# Autodesk Inventor assembly: Enclosure02
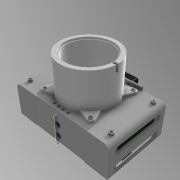
[picture p0: Inventor's stored thumbnail of the model, 180x180]
Saved by Autodesk Inventor 2013 (Build 170138000, 138)
## iProperties
Created: 2014-04-13
Part Number: Enclosure02
Document SubType Name: Assembly
Designer: spichelh
Author: spichelh
## Documents named in this file (22)
- C:\Users\spichelh\Documents\GitHub\beta-hardware\Enclosure\Version 002\Enclosure02.iam
- C:\Users\spichelh\Documents\GitHub\beta-hardware\Enclosure\Version 002\PCB01.ipt
- C:\Users\spichelh\Documents\GitHub\beta-hardware\Enclosure\Version 002\Microzed01.ipt
- C:\Users\spichelh\Documents\GitHub\beta-hardware\Enclosure\Version 002\AddonPCB01.ipt
- C:\Users\spichelh\Documents\GitHub\beta-hardware\Enclosure\Version 002\Enclosure-Backplate01.ipt
- C:\Users\spichelh\Documents\GitHub\beta-hardware\Enclosure\Version 002\KAC12040.ipt
- C:\Users\spichelh\Documents\GitHub\beta-hardware\Enclosure\Version 002\IRGlass.ipt
- C:\Users\spichelh\Documents\GitHub\beta-hardware\Enclosure\Version 002\Cooler.ipt
- C:\Users\spichelh\Documents\GitHub\beta-hardware\Enclosure\Version 002\Nikon Mount 02.ipt
- C:\Users\spichelh\Documents\GitHub\beta-hardware\Enclosure\Version 002\IOModulePlate01.ipt
- C:\Users\spichelh\Documents\GitHub\beta-hardware\Enclosure\Version 002\PCBModuleLeft01.ipt
- C:\Users\spichelh\Documents\GitHub\beta-hardware\Enclosure\Version 002\IOModulePlate02.ipt
- C:\Users\spichelh\Documents\GitHub\beta-hardware\Enclosure\Version 002\IOModulePlate03.ipt
- C:\Users\spichelh\Documents\GitHub\beta-hardware\Enclosure\Version 002\PCBModuleRight01.ipt
- C:\Users\spichelh\Documents\GitHub\beta-hardware\Enclosure\Version 002\LensBase02.ipt
- C:\Users\spichelh\Documents\GitHub\beta-hardware\Enclosure\Version 002\HexSaver01.ipt
- C:\Users\spichelh\Documents\GitHub\beta-hardware\Enclosure\Version 002\Enclosure03.ipt
- C:\Users\spichelh\Documents\Inventor\Content Center Files\R2013\en-US\ANSI B18.3.1M(1)\ANSI B18.3.1M - M2,5x0,45 x 16(2).ipt
- C:\Users\spichelh\Documents\Inventor\Content Center Files\R2013\en-US\ANSI B18.3.1M(1)\ANSI B18.3.1M - M2,5x0,45 x 35(2).ipt
- C:\Users\spichelh\Documents\GitHub\beta-hardware\Enclosure\Version 002\LensBaseTop01.ipt
- C:\Users\spichelh\Documents\Inventor\Content Center Files\R2013\en-US\ANSI B18.6.3(00)\ANSI B18.6.3 - 3-48 UNC - 0,25(32).ipt
- C:\Users\spichelh\Documents\GitHub\beta-hardware\Enclosure\Version 002\Unmate01.ipt
## Components (34 placed, 21 different names)
1. Enclosure03:1 — Flush:26, Mate:33, Mate:34, Mate:38, Flush:40, Mate:39, Insert:9, Insert:10, Insert:11, Insert:13, Insert:14, Insert:26, Insert:27, Insert:28, Insert:29
2. PCB01:1 — Mate:1, Flush:1, Flush:2, Flush:21, Flush:22, Flush:23, Insert:1, Mate:37, Flush:41, Flush:42, Mate:40, Mate:41, Mate:42, Mate:43, Mate:44, Mate:45, Insert:15, Mate:46, Mate:47, Insert:16, Mate:48, Mate:49, Insert:17, Mate:64, Mate:62, Mate:65, Mate:58, Mate:56
3. Microzed01:1 — Mate:1, Flush:1, Flush:2, Flush:22, Flush:24, Flush:27, Mate:36
4. AddonPCB01:1 — Flush:24, Flush:27, Mate:36
5. Enclosure-Backplate01:1 — Mate:38, Flush:40
6. KAC12040:1 — Mate:37
7. IRGlass:1 — Mate:50, Mate:51, Mate:52
8. Cooler:1 — Mate:35, Flush:43, Flush:44, Mate:67, Mate:68, Mate:69
9. Nikon Mount 02:1 — Mate:31, Mate:32, Insert:3, Mate:50, Mate:51, Mate:52, Insert:18, Insert:19, Insert:20, Insert:21
10. LensBase02:1 — Mate:31, Mate:32, Insert:1, Flush:26, Mate:33, Mate:34, Insert:3, Mate:35, Flush:43, Flush:44, Flush:45
11. IOModulePlate01:1 — Insert:13, Insert:14
12. PCBModuleLeft01:1 — Flush:21, Flush:23, Mate:62
13. PCBModuleRight01:1 — Flush:41, Flush:42, Mate:40
14. IOModulePlate02:1 — Insert:11
15. IOModulePlate03:1 — Insert:9, Insert:10
16. HexSaver01:1 — Mate:41, Mate:42, Mate:43
17. HexSaver01:2 — Mate:44, Mate:45, Insert:15
18. HexSaver01:3 — Mate:46, Mate:47, Insert:16
19. HexSaver01:4 — Mate:48, Mate:49, Insert:17
20. Broached Socket Head Cap Screw - Metric M2,5x0,45 x 16:1 — Insert:18
21. Broached Socket Head Cap Screw - Metric M2,5x0,45 x 16:2 — Insert:19
22. Broached Socket Head Cap Screw - Metric M2,5x0,45 x 16:3 — Insert:20
23. Broached Socket Head Cap Screw - Metric M2,5x0,45 x 16:4 — Insert:21
24. LensBaseTop01:1 — Flush:45, Mate:53, Mate:54, Mate:67, Mate:68, Mate:69
25. Cross Recessed 100° Flat Countersunk Head Machine Screw - Type I - Inch 3-48 UNC x 0,25:2 — Mate:53
26. Cross Recessed 100° Flat Countersunk Head Machine Screw - Type I - Inch 3-48 UNC x 0,25:1 — Mate:54
27. Broached Socket Head Cap Screw - Metric M2,5x0,45 x 35:5 — Insert:26, Mate:55
28. Broached Socket Head Cap Screw - Metric M2,5x0,45 x 35:6 — Insert:27, Mate:59
29. Broached Socket Head Cap Screw - Metric M2,5x0,45 x 35:7 — Insert:28, Mate:66
30. Broached Socket Head Cap Screw - Metric M2,5x0,45 x 35:8 — Insert:29, Mate:57
31. Unmate01:1 — Mate:55, Mate:56
32. Unmate01:2 — Mate:57, Mate:58
33. Unmate01:3 — Mate:59, Mate:64
34. Unmate01:4 — Mate:65, Mate:66
## Relationships (69: Mate 37, Insert 18, Flush 14)
- Mate:1 (5 mm): PCB01:1 ↔ Microzed01:1
- Flush:1: PCB01:1 ↔ Microzed01:1
- Flush:2: PCB01:1 ↔ Microzed01:1
- Flush:21: PCB01:1 ↔ PCBModuleLeft01:1
- Flush:22: PCB01:1 ↔ Microzed01:1
- Flush:23: PCB01:1 ↔ PCBModuleLeft01:1
- Flush:24: Microzed01:1 ↔ AddonPCB01:1
- Mate:31: Nikon Mount 02:1 ↔ LensBase02:1
- Mate:32: Nikon Mount 02:1 ↔ LensBase02:1
- Insert:1: PCB01:1 ↔ LensBase02:1
- Flush:26: Enclosure03:1 ↔ LensBase02:1
- Mate:33: Enclosure03:1 ↔ LensBase02:1
- Mate:34: Enclosure03:1 ↔ LensBase02:1
- Insert:3: Nikon Mount 02:1 ↔ LensBase02:1
- Mate:35: Cooler:1 ↔ LensBase02:1
- Flush:27: Microzed01:1 ↔ AddonPCB01:1
- Mate:36 (10 mm): Microzed01:1 ↔ AddonPCB01:1
- Mate:37: PCB01:1 ↔ KAC12040:1
- Mate:38 (-1 mm): Enclosure03:1 ↔ Enclosure-Backplate01:1
- Flush:40: Enclosure03:1 ↔ Enclosure-Backplate01:1
- Mate:39: Enclosure03:1
- Flush:41: PCB01:1 ↔ PCBModuleRight01:1
- Flush:42: PCB01:1 ↔ PCBModuleRight01:1
- Mate:40 (6 mm): PCB01:1 ↔ PCBModuleRight01:1
- Insert:9: Enclosure03:1 ↔ IOModulePlate03:1
- Insert:10: Enclosure03:1 ↔ IOModulePlate03:1
- Insert:11: Enclosure03:1 ↔ IOModulePlate02:1
- Insert:13: Enclosure03:1 ↔ IOModulePlate01:1
- Insert:14: Enclosure03:1 ↔ IOModulePlate01:1
- Mate:41: PCB01:1 ↔ HexSaver01:1
- Mate:42: PCB01:1 ↔ HexSaver01:1
- Mate:43: PCB01:1 ↔ HexSaver01:1
- Mate:44: PCB01:1 ↔ HexSaver01:2
- Mate:45: PCB01:1 ↔ HexSaver01:2
- Insert:15: PCB01:1 ↔ HexSaver01:2
- Mate:46: PCB01:1 ↔ HexSaver01:3
- Mate:47: PCB01:1 ↔ HexSaver01:3
- Insert:16: PCB01:1 ↔ HexSaver01:3
- Mate:48: PCB01:1 ↔ HexSaver01:4
- Mate:49: PCB01:1 ↔ HexSaver01:4
- Insert:17: PCB01:1 ↔ HexSaver01:4
- Mate:50: IRGlass:1 ↔ Nikon Mount 02:1
- Mate:51 (0.5 mm): IRGlass:1 ↔ Nikon Mount 02:1
- Mate:52 (0.5 mm): IRGlass:1 ↔ Nikon Mount 02:1
- Flush:43: Cooler:1 ↔ LensBase02:1
- Flush:44: Cooler:1 ↔ LensBase02:1
- Flush:45: LensBase02:1 ↔ LensBaseTop01:1
- Mate:55: Broached Socket Head Cap Screw - Metric M2,5x0,45 x 35:5 ↔ Unmate01:1
- Mate:56: PCB01:1 ↔ Unmate01:1
- Mate:57: Broached Socket Head Cap Screw - Metric M2,5x0,45 x 35:8 ↔ Unmate01:2
- Mate:58: PCB01:1 ↔ Unmate01:2
- Mate:59: Broached Socket Head Cap Screw - Metric M2,5x0,45 x 35:6 ↔ Unmate01:3
- Mate:62 (6 mm): PCB01:1 ↔ PCBModuleLeft01:1
- Mate:64: PCB01:1 ↔ Unmate01:3
- Mate:65: PCB01:1 ↔ Unmate01:4
- Mate:66: Broached Socket Head Cap Screw - Metric M2,5x0,45 x 35:7 ↔ Unmate01:4
- Mate:67: Cooler:1 ↔ LensBaseTop01:1
- Mate:68: Cooler:1 ↔ LensBaseTop01:1
- Mate:69: Cooler:1 ↔ LensBaseTop01:1
- Insert:18: Nikon Mount 02:1 ↔ Broached Socket Head Cap Screw - Metric M2,5x0,45 x 16:1
- Insert:19: Nikon Mount 02:1 ↔ Broached Socket Head Cap Screw - Metric M2,5x0,45 x 16:2
- Insert:20: Nikon Mount 02:1 ↔ Broached Socket Head Cap Screw - Metric M2,5x0,45 x 16:3
- Insert:21: Nikon Mount 02:1 ↔ Broached Socket Head Cap Screw - Metric M2,5x0,45 x 16:4
- Mate:53: LensBaseTop01:1 ↔ Cross Recessed 100° Flat Countersunk Head Machine Screw - Type I - Inch 3-48 UNC x 0,25:2
- Mate:54: LensBaseTop01:1 ↔ Cross Recessed 100° Flat Countersunk Head Machine Screw - Type I - Inch 3-48 UNC x 0,25:1
- Insert:26: Enclosure03:1 ↔ Broached Socket Head Cap Screw - Metric M2,5x0,45 x 35:5
- Insert:27: Enclosure03:1 ↔ Broached Socket Head Cap Screw - Metric M2,5x0,45 x 35:6
- Insert:28: Enclosure03:1 ↔ Broached Socket Head Cap Screw - Metric M2,5x0,45 x 35:7
- Insert:29: Enclosure03:1 ↔ Broached Socket Head Cap Screw - Metric M2,5x0,45 x 35:8
